# Autodesk Inventor assembly: rimAssembly
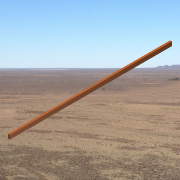
[picture p0: Inventor's stored thumbnail of the model, 180x180]
Saved by Autodesk Inventor 2014 SP1 (Build 180222100, 222)
## iProperties
Created: 2013-12-03
Part Number: rimAssembly
Document SubType Name: Assembly
Designer: Dave
Author: Dave
## Documents named in this file (3)
- C:\Users\Dave\Desktop\hera-cad\support\rimAssembly.iam
- C:\Users\Dave\Desktop\hera-cad\support\rimHoriz.ipt
- C:\Users\Dave\Desktop\hera-cad\support\rimIntermediateSparHolder.ipt
## Components (2 placed, 2 different names)
1. rimHoriz:1 — Insert:1, Angle:1
2. rimIntermediateSparHolder:1 — Insert:1, Angle:1
## Relationships (2: Insert 1, Angle 1)
- Insert:1: rimHoriz:1 ↔ rimIntermediateSparHolder:1
- Angle:1 (37.26 deg): rimHoriz:1 ↔ rimIntermediateSparHolder:1
